# Autodesk Inventor assembly: Wheel
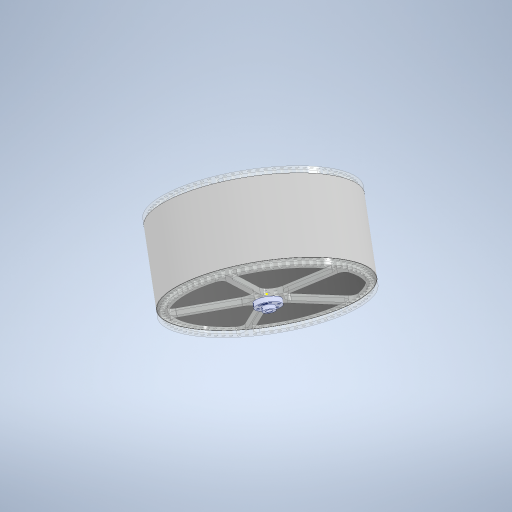
[picture p0: Inventor's stored thumbnail of the model, 512x512]
Saved by Autodesk Inventor 2024 (Build 280153000, 153)
## iProperties
Created: 2022-02-01
Part Number: Wheel
Document SubType Name: Assembly
Designer: gnzak
Author: gnzak
## Documents named in this file (4)
- C:\Users\rosam\OneDrive\Documents\github_latest\Hardware\Tablet-Rig\Assemblies\Wheel.iam
- C:\Users\rosam\OneDrive\Documents\github_latest\Hardware\Tablet-Rig\Parts\Spokes\spokes.ipt
- C:\Users\rosam\OneDrive\Documents\github_latest\Hardware\Tablet-Rig\Parts\Pololu 1993\Pololu 1993.ipt
- C:\Users\rosam\OneDrive\Documents\github_latest\Hardware\Tablet-Rig\Parts\Track\Polycarbonate Track.ipt
## Components (5 placed, 3 different names)
1. spokes:1 — Mate:9
2. Pololu 1993:1
3. Polycarbonate Track:1 — Mate:8, Mate:9
4. spokes:2 — Mate:8, Mate:10
5. Pololu 1993:2 — Mate:10
## Relationships (9: Mate 8, Flush 1)
- [Mate]: spokes:1 ↔ Pololu 1993:1
- [Mate]: spokes:1 ↔ Pololu 1993:1
- [Mate]: spokes:1 ↔ Polycarbonate Track:1
- [Mate]: Polycarbonate Track:1 ↔ spokes:2
- [Mate]: spokes:2 ↔ Pololu 1993:2
- [Flush]: spokes:1 ↔ spokes:2
- Mate:8: Polycarbonate Track:1 ↔ spokes:2
- Mate:9: spokes:1 ↔ Polycarbonate Track:1
- Mate:10: spokes:2 ↔ Pololu 1993:2
